# Autodesk Inventor assembly: BC-100003_Base maior
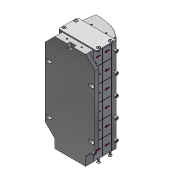
[picture p0: Inventor's stored thumbnail of the model, 180x180]
Saved by Autodesk Inventor 2016 (Build 200138000, 138)
## iProperties
Created: 2015-09-23
Part Number: BC-100003_Base maior
Document SubType Name: Assembly
Designer: Reinaldo.Basílio
Mass: 37161.3 g
Surface Area: 6721.8 cm^2
Volume: 5243.53 cm^3
Density: 7.08707 g/cm^3
Author: Reinaldo.Basílio
## Documents named in this file (8)
- D:\ARQ\Basilio\LNLS-2\Anel\Dipolos\BC-3T\Dipolo 3T e 1T\Prototipo 1\Projeto Mecanico\BC-100001-A-Inf.iam
- D:\ARQ\Basilio\LNLS-2\Anel\Dipolos\BC-3T\Dipolo 3T e 1T\Prototipo 1\Projeto Mecanico\BC-100002.iam
- D:\ARQ\Basilio\LNLS-2\Anel\Dipolos\BC-3T\Dipolo 3T e 1T\Prototipo 1\Projeto Mecanico\BC-10003-A.ipt
- D:\ARQ\Basilio\LNLS-2\Anel\Dipolos\BC-3T\Dipolo 3T e 1T\Prototipo 1\Projeto Mecanico\BC-10004.ipt
- D:\ARQ\Basilio\LNLS-2\Anel\Dipolos\BC-3T\Dipolo 3T e 1T\Prototipo 1\Projeto Mecanico\BC-10017.ipt
- D:\ARQ\Basilio\LNLS-2\Anel\Dipolos\BC-3T\Dipolo 3T e 1T\Prototipo 1\Projeto Mecanico\BC-10024.ipt
- D:\ARQ\Basilio\LNLS-2\Anel\Dipolos\BC-3T\Dipolo 3T e 1T\Prototipo 1\Projeto Mecanico\Parafusos\DIN 912 - M6x20.ipt
- D:\ARQ\Basilio\LNLS-2\Anel\Dipolos\BC-3T\Dipolo 3T e 1T\Prototipo 1\Projeto Mecanico\Parafusos\DIN 7991 - M5x12.ipt
## Components (35 placed, 7 different names)
1. BC-10003-A:1 — Flush:10, Mate:4, Mate:5, Flush:12, Mate:6, Flush:13, Insert:1, Insert:4
2. BC-100002:1 [sub-assembly] — Mate:2, Flush:7, Flush:11, Mate:6
3. BC-10004:1 — Mate:2, Flush:7, Flush:11, Flush:12, Flush:13, Insert:2, Insert:3
4. BC-10017:1 — Insert:1, Insert:2, Insert:5, Insert:8, Insert:9, Insert:10, Insert:11, Insert:12, Insert:13, Insert:14, Insert:15, Insert:16, Insert:17, Insert:18
5. BC-10017:2 — Insert:3, Insert:4, Insert:6, Insert:7, Insert:19, Insert:20, Insert:21, Insert:22, Insert:23, Insert:24, Insert:25, Insert:26, Insert:27, Insert:28
6. BC-10024:1 — Insert:5, Insert:6, Insert:29, Insert:30, Insert:31, Insert:32
7. BC-10024:2 — Insert:7, Insert:8, Insert:33, Insert:34, Insert:35, Insert:36
8. DIN 912 - Parafuso Allen com cabeça (Inox) M6x20:1 — Insert:9
9. DIN 912 - Parafuso Allen com cabeça (Inox) M6x20:2 — Insert:10
10. DIN 912 - Parafuso Allen com cabeça (Inox) M6x20:3 — Insert:11
11. DIN 912 - Parafuso Allen com cabeça (Inox) M6x20:4 — Insert:12
12. DIN 912 - Parafuso Allen com cabeça (Inox) M6x20:5 — Insert:13
13. DIN 912 - Parafuso Allen com cabeça (Inox) M6x20:6 — Insert:14
14. DIN 912 - Parafuso Allen com cabeça (Inox) M6x20:7 — Insert:15
15. DIN 912 - Parafuso Allen com cabeça (Inox) M6x20:8 — Insert:16
16. DIN 912 - Parafuso Allen com cabeça (Inox) M6x20:9 — Insert:17
17. DIN 912 - Parafuso Allen com cabeça (Inox) M6x20:10 — Insert:18
18. DIN 912 - Parafuso Allen com cabeça (Inox) M6x20:11 — Insert:19
19. DIN 912 - Parafuso Allen com cabeça (Inox) M6x20:12 — Insert:20
20. DIN 912 - Parafuso Allen com cabeça (Inox) M6x20:13 — Insert:21
21. DIN 912 - Parafuso Allen com cabeça (Inox) M6x20:14 — Insert:22
22. DIN 912 - Parafuso Allen com cabeça (Inox) M6x20:15 — Insert:23
23. DIN 912 - Parafuso Allen com cabeça (Inox) M6x20:16 — Insert:24
24. DIN 912 - Parafuso Allen com cabeça (Inox) M6x20:17 — Insert:25
25. DIN 912 - Parafuso Allen com cabeça (Inox) M6x20:18 — Insert:26
26. DIN 912 - Parafuso Allen com cabeça (Inox) M6x20:19 — Insert:27
27. DIN 912 - Parafuso Allen com cabeça (Inox) M6x20:20 — Insert:28
28. DIN 7991 - Parafuso Allen com cabeça chata (inox) M5x12:1 — Insert:29
29. DIN 7991 - Parafuso Allen com cabeça chata (inox) M5x12:2 — Insert:30
30. DIN 7991 - Parafuso Allen com cabeça chata (inox) M5x12:3 — Insert:31
31. DIN 7991 - Parafuso Allen com cabeça chata (inox) M5x12:4 — Insert:32
32. DIN 7991 - Parafuso Allen com cabeça chata (inox) M5x12:5 — Insert:33
33. DIN 7991 - Parafuso Allen com cabeça chata (inox) M5x12:6 — Insert:34
34. DIN 7991 - Parafuso Allen com cabeça chata (inox) M5x12:7 — Insert:35
35. DIN 7991 - Parafuso Allen com cabeça chata (inox) M5x12:8 — Insert:36
## Relationships (45: Insert 36, Flush 5, Mate 4)
- Mate:2: BC-100002:1 ↔ BC-10004:1
- Flush:7: BC-100002:1 ↔ BC-10004:1
- Flush:10: BC-10003-A:1
- Mate:4: BC-10003-A:1
- Mate:5 (-57.5 mm): BC-10003-A:1
- Flush:11: BC-100002:1 ↔ BC-10004:1
- Flush:12: BC-10003-A:1 ↔ BC-10004:1
- Mate:6: BC-10003-A:1 ↔ BC-100002:1
- Flush:13: BC-10003-A:1 ↔ BC-10004:1
- Insert:1: BC-10003-A:1 ↔ BC-10017:1
- Insert:2: BC-10004:1 ↔ BC-10017:1
- Insert:3: BC-10004:1 ↔ BC-10017:2
- Insert:4: BC-10003-A:1 ↔ BC-10017:2
- Insert:5: BC-10017:1 ↔ BC-10024:1
- Insert:6: BC-10017:2 ↔ BC-10024:1
- Insert:7: BC-10017:2 ↔ BC-10024:2
- Insert:8: BC-10017:1 ↔ BC-10024:2
- Insert:9: BC-10017:1 ↔ DIN 912 - Parafuso Allen com cabeça (Inox) M6x20:1
- Insert:10: BC-10017:1 ↔ DIN 912 - Parafuso Allen com cabeça (Inox) M6x20:2
- Insert:11: BC-10017:1 ↔ DIN 912 - Parafuso Allen com cabeça (Inox) M6x20:3
- Insert:12: BC-10017:1 ↔ DIN 912 - Parafuso Allen com cabeça (Inox) M6x20:4
- Insert:13: BC-10017:1 ↔ DIN 912 - Parafuso Allen com cabeça (Inox) M6x20:5
- Insert:14: BC-10017:1 ↔ DIN 912 - Parafuso Allen com cabeça (Inox) M6x20:6
- Insert:15: BC-10017:1 ↔ DIN 912 - Parafuso Allen com cabeça (Inox) M6x20:7
- Insert:16: BC-10017:1 ↔ DIN 912 - Parafuso Allen com cabeça (Inox) M6x20:8
- Insert:17: BC-10017:1 ↔ DIN 912 - Parafuso Allen com cabeça (Inox) M6x20:9
- Insert:18: BC-10017:1 ↔ DIN 912 - Parafuso Allen com cabeça (Inox) M6x20:10
- Insert:19: BC-10017:2 ↔ DIN 912 - Parafuso Allen com cabeça (Inox) M6x20:11
- Insert:20: BC-10017:2 ↔ DIN 912 - Parafuso Allen com cabeça (Inox) M6x20:12
- Insert:21: BC-10017:2 ↔ DIN 912 - Parafuso Allen com cabeça (Inox) M6x20:13
- Insert:22: BC-10017:2 ↔ DIN 912 - Parafuso Allen com cabeça (Inox) M6x20:14
- Insert:23: BC-10017:2 ↔ DIN 912 - Parafuso Allen com cabeça (Inox) M6x20:15
- Insert:24: BC-10017:2 ↔ DIN 912 - Parafuso Allen com cabeça (Inox) M6x20:16
- Insert:25: BC-10017:2 ↔ DIN 912 - Parafuso Allen com cabeça (Inox) M6x20:17
- Insert:26: BC-10017:2 ↔ DIN 912 - Parafuso Allen com cabeça (Inox) M6x20:18
- Insert:27: BC-10017:2 ↔ DIN 912 - Parafuso Allen com cabeça (Inox) M6x20:19
- Insert:28: BC-10017:2 ↔ DIN 912 - Parafuso Allen com cabeça (Inox) M6x20:20
- Insert:29: BC-10024:1 ↔ DIN 7991 - Parafuso Allen com cabeça chata (inox) M5x12:1
- Insert:30: BC-10024:1 ↔ DIN 7991 - Parafuso Allen com cabeça chata (inox) M5x12:2
- Insert:31: BC-10024:1 ↔ DIN 7991 - Parafuso Allen com cabeça chata (inox) M5x12:3
- Insert:32: BC-10024:1 ↔ DIN 7991 - Parafuso Allen com cabeça chata (inox) M5x12:4
- Insert:33: BC-10024:2 ↔ DIN 7991 - Parafuso Allen com cabeça chata (inox) M5x12:5
- Insert:34: BC-10024:2 ↔ DIN 7991 - Parafuso Allen com cabeça chata (inox) M5x12:6
- Insert:35: BC-10024:2 ↔ DIN 7991 - Parafuso Allen com cabeça chata (inox) M5x12:7
- Insert:36: BC-10024:2 ↔ DIN 7991 - Parafuso Allen com cabeça chata (inox) M5x12:8
